# Autodesk Inventor assembly: KB33-046-001 - Ходовая часть
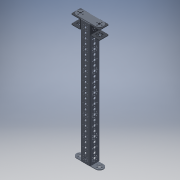
[picture p0: Inventor's stored thumbnail of the model, 180x180]
Saved by Autodesk Inventor 2019 (Build 230136000, 136)
## iProperties
Created: 2021-06-08
Part Number: KB33-046-001 - Ходовая часть
Material: Типовые
Document SubType Name: Assembly
Designer: Петров Иван
Author: Петров Иван
## Documents named in this file (5)
- E:\IVAN\Ivan_desktop\Kvantorium\Projects\RoboPatrol\design\KB33-046-002 - Рама.iam
- E:\IVAN\Ivan_desktop\Kvantorium\Projects\RoboPatrol\design\KB33-046-001-001 - Основание.ipt
- E:\IVAN\Ivan_desktop\Kvantorium\Projects\RoboPatrol\design\standart_components\Tetrix\ftc-tetrix-kit-of-parts-1.snapshot.34\MAX Channels\416mm Channel.ipt
- E:\IVAN\Ivan_desktop\Kvantorium\Projects\RoboPatrol\design\standart_components\Tetrix\ftc-tetrix-kit-of-parts-1.snapshot.34\Brackets\MAX Flat Bracket.ipt
- E:\IVAN\Ivan_desktop\Kvantorium\Projects\RoboPatrol\design\standart_components\Tetrix\ftc-tetrix-kit-of-parts-1.snapshot.34\MAX Channels\32mm Channel.ipt
## Components (6 placed, 4 different names)
1. KB33-046-001-001 - Основание:1
2. 416mm Channel:1 — Mate:1, Mate:2, Mate:3, Mate:4, Mate:5, Mate:7, Mate:8
3. MAX Flat Bracket:1 — Mate:6, Mate:9
4. MAX Flat Bracket:2
5. 32mm Channel:1 — Mate:4, Mate:5, Mate:6
6. 32mm Channel:2 — Mate:7, Mate:8, Mate:9
## Relationships (9: Mate 9)
- Mate:1: 416mm Channel:1
- Mate:2: 416mm Channel:1
- Mate:3: 416mm Channel:1
- Mate:4: 416mm Channel:1 ↔ 32mm Channel:1
- Mate:5: 416mm Channel:1 ↔ 32mm Channel:1
- Mate:6: MAX Flat Bracket:1 ↔ 32mm Channel:1
- Mate:7: 416mm Channel:1 ↔ 32mm Channel:2
- Mate:8: 416mm Channel:1 ↔ 32mm Channel:2
- Mate:9: MAX Flat Bracket:1 ↔ 32mm Channel:2
